# Autodesk Inventor assembly: MUSAB ASSEMPLY
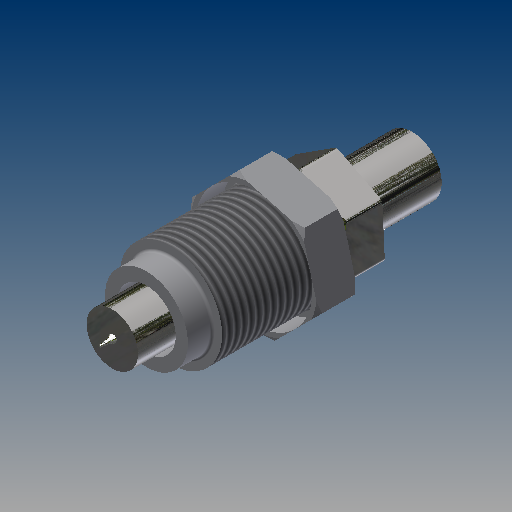
[picture p0: Inventor's stored thumbnail of the model, 512x512]
Saved by Autodesk Inventor 2021 (Build 250183000, 183)
## iProperties
Created: 2017-09-15
Part Number: MUSAB ASSEMPLY
Document SubType Name: Assembly
Designer: Amer Mohia
Author: Amer Mohia
## Documents named in this file (8)
- C:\Users\Angelos\Documents\ΔεΝ_τΕλΕιΩνΟυΜε_ΠοΤε\MUSAB ASSEMPLY.iam
- C:\Users\Angelos\Documents\ΔεΝ_τΕλΕιΩνΟυΜε_ΠοΤε\MUSAB1.ipt
- C:\Users\Angelos\Documents\ΔεΝ_τΕλΕιΩνΟυΜε_ΠοΤε\Musab7.ipt
- C:\Users\Angelos\Documents\ΔεΝ_τΕλΕιΩνΟυΜε_ΠοΤε\MUSAB5.ipt
- C:\Users\Angelos\Documents\ΔεΝ_τΕλΕιΩνΟυΜε_ΠοΤε\MUSAB6.ipt
- C:\Users\Angelos\Documents\ΔεΝ_τΕλΕιΩνΟυΜε_ΠοΤε\Musab4.ipt
- C:\Users\Angelos\Documents\ΔεΝ_τΕλΕιΩνΟυΜε_ΠοΤε\Part4.ipt
- C:\Users\Angelos\Documents\ΔεΝ_τΕλΕιΩνΟυΜε_ΠοΤε\MUSAB2.ipt
## Components (7 placed, 7 different names)
1. MUSAB1:1 — Mate:1, Mate:2, Mate:5, Mate:6, Mate:11, Mate:17, Mate:18
2. Musab7:1 — Mate:1, Mate:2
3. MUSAB5:1 — Mate:5, Mate:7, Mate:16, Mate:17, Mate:18
4. MUSAB6:1 — Mate:6, Mate:9, Mate:10, Mate:15, Mate:16
5. Musab4:1 — Mate:8, Mate:9, Mate:10, Mate:14, Insert:1
6. Part4:1 — Mate:7, Mate:8, Insert:1
7. MUSAB2:1 — Mate:11, Mate:14, Mate:15
## Relationships (15: Mate 14, Insert 1)
- Mate:1: MUSAB1:1 ↔ Musab7:1
- Mate:2: MUSAB1:1 ↔ Musab7:1
- Mate:5: MUSAB1:1 ↔ MUSAB5:1
- Mate:6: MUSAB1:1 ↔ MUSAB6:1
- Mate:7: MUSAB5:1 ↔ Part4:1
- Mate:8: Musab4:1 ↔ Part4:1
- Mate:9: MUSAB6:1 ↔ Musab4:1
- Mate:10: MUSAB6:1 ↔ Musab4:1
- Mate:11: MUSAB1:1 ↔ MUSAB2:1
- Mate:14: Musab4:1 ↔ MUSAB2:1
- Mate:15: MUSAB6:1 ↔ MUSAB2:1
- Mate:16: MUSAB5:1 ↔ MUSAB6:1
- Mate:17: MUSAB1:1 ↔ MUSAB5:1
- Mate:18: MUSAB1:1 ↔ MUSAB5:1
- Insert:1 (0.3 mm): Musab4:1 ↔ Part4:1
